# Autodesk Inventor assembly: CP3x3
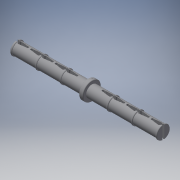
[picture p0: Inventor's stored thumbnail of the model, 180x180]
Saved by Autodesk Inventor 2019.3 (Build 233278000, 278)
## iProperties
Created: 2019-02-05
Part Number: CP3x3
Document SubType Name: Assembly
Designer: Varga Daniel
Author: Varga Daniel
## Documents named in this file (6)
- C:\!_Dani\!_cloud\OneDrive\!_munka\Revolution\RevvyDemoKit\Structural parts\Connetor Pins\CP1+x1+\CP3x3.iam
- C:\!_Dani\!_cloud\OneDrive\!_munka\Revolution\RevvyDemoKit\Structural parts\Connetor Pins\Connector_pin_collar.ipt
- C:\!_Dani\!_cloud\OneDrive\!_munka\Revolution\RevvyDemoKit\Structural parts\Connetor Pins\Connector_pin_stick.ipt
- C:\!_Dani\!_cloud\OneDrive\!_munka\Revolution\RevvyDemoKit\Structural parts\Connetor Pins\Connector_pin_stack_stick.ipt
- C:\!_Dani\!_cloud\OneDrive\!_munka\Revolution\RevvyDemoKit\Structural parts\Connetor Pins\Connector_pin_base.ipt
- C:\!_Dani\!_cloud\OneDrive\!_munka\Revolution\RevvyDemoKit\Structural parts\Connetor Pins\CP1+x1+.iam
## Components (8 placed, 3 different names)
1. Connector_pin_collar:1 — Mate:1, Mate:2, Mate:3, Mate:6, Mate:7
2. Connector_pin_stick:1 — Mate:2, Mate:3, Flush:1, Angle:1, Mate:10, Mate:11, Angle:3
3. Connector_pin_collar:2 — Mate:6, Mate:7
4. Connector_pin_stick:2 — Flush:1, Mate:8, Mate:9, Angle:2
5. Connector_pin_stack_stick:2 — Mate:10, Mate:11, Angle:3
6. Connector_pin_stack_stick:3
7. Connector_pin_stack_stick:1 — Mate:8, Mate:9, Angle:2
8. Connector_pin_stack_stick:4
## Component patterns: (2 elements, first: Connector_pin_stack_stick:2), (2 elements, first: Connector_pin_stack_stick:1)
## Relationships (15: Mate 11, Angle 3, Flush 1)
- Mate:1: Connector_pin_collar:1
- Mate:2: Connector_pin_collar:1 ↔ Connector_pin_stick:1
- Mate:3: Connector_pin_collar:1 ↔ Connector_pin_stick:1
- [Mate]: Connector_pin_collar:2 ↔ Connector_pin_stick:2
- [Mate]: Connector_pin_collar:2 ↔ Connector_pin_stick:2
- Mate:6: Connector_pin_collar:1 ↔ Connector_pin_collar:2
- Mate:7: Connector_pin_collar:1 ↔ Connector_pin_collar:2
- Flush:1: Connector_pin_stick:1 ↔ Connector_pin_stick:2
- Angle:1 (0 deg): Connector_pin_stick:1
- Mate:8: Connector_pin_stick:2 ↔ Connector_pin_stack_stick:1
- Mate:9: Connector_pin_stick:2 ↔ Connector_pin_stack_stick:1
- Angle:2 (0 deg): Connector_pin_stick:2 ↔ Connector_pin_stack_stick:1
- Mate:10: Connector_pin_stick:1 ↔ Connector_pin_stack_stick:2
- Mate:11: Connector_pin_stick:1 ↔ Connector_pin_stack_stick:2
- Angle:3 (0 deg): Connector_pin_stick:1 ↔ Connector_pin_stack_stick:2
## Named parameters: d3_d1 = 0 mm, d4_d2 = 0 mm, Collar_thickness = 1.726 mm, Pin_diameter = 4.95 mm, Collar_diameter = 7.5 mm, Pin_overall_length = 19.976 mm, Pin_inner_length = 8.425 mm, Upper_ring_diameter = 5.5 mm, Upper_ring_thickness = 0.7 mm, Pin_stack_height = 10.125 mm, Stack_num_left = 2, Stack_num_right = 2
